# Autodesk Inventor assembly: BodyStructure
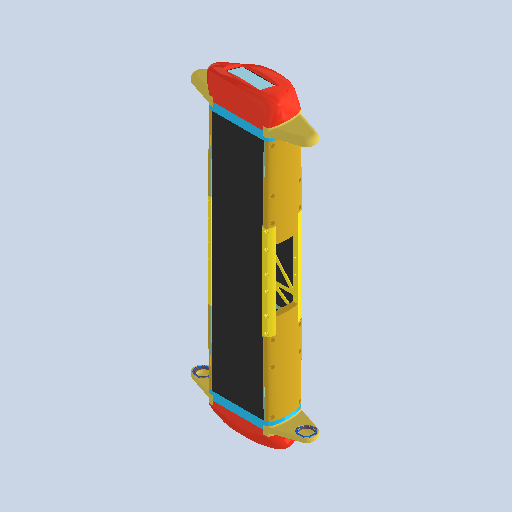
[picture p0: Inventor's stored thumbnail of the model, 512x512]
Saved by Autodesk Inventor 2023 (Build 270158000, 158)
## iProperties
Created: 2022-01-14
Part Number: BodyStructure
Document SubType Name: Assembly
Designer: Jochen
Author: Jochen
## Documents named in this file (11)
- D:\Projects\Lisbeth\CAD\BodyStructure.iam
- D:\Projects\Lisbeth\CAD\Body\BodyStructure Side.ipt
- D:\Projects\Lisbeth\CAD\Body\BodyStructure HipSupport.ipt
- D:\Projects\Lisbeth\CAD\Body\BodyStructure Centre Top.ipt
- D:\Projects\Lisbeth\CAD\Common\Bearing\bearing_27_20_4 s61704-2rsr.ipt
- D:\Projects\Lisbeth\CAD\Body\BodyCover.ipt
- D:\Projects\Lisbeth\CAD\Common\Accessories\Battery Pack.ipt
- D:\Projects\Lisbeth\CAD\Body\BodyStructure Head.ipt
- D:\Projects\Lisbeth\CAD\Body\BodyStructure Tail.ipt
- D:\Projects\Lisbeth\CAD\Common\Accessories\Adafruit 2.4 OLED display.ipt
- D:\Projects\Lisbeth\CAD\Body\BodyStructure Plate.ipt
## Components (24 placed, 9 different names)
1. BodyHipSupport:1 — Mate:38, Mate:39, Mate:230, Mate:231
2. BodyHipSupport:2 — Mate:44, Mate:45, Mate:226, Mate:227
3. BodyHipSupport:3 — Mate:42, Mate:43, Mate:188, Mate:189
4. BodyHipSupport:4 — Mate:40, Mate:41, Mate:147, Mate:148
5. bearing_27_20_4 s61704-2rsr:1 — Mate:38, Mate:39
6. bearing_27_20_4 s61704-2rsr:2 — Mate:44, Mate:45
7. bearing_27_20_4 s61704-2rsr:3 — Mate:40, Mate:41
8. bearing_27_20_4 s61704-2rsr:4 — Mate:42, Mate:43
9. BodyCover:1 — Mate:217, Mate:219
10. BodyCover:2 — Angle:1, Mate:202, Mate:204
11. Battery Pack 59x31x21:1 — Angle:1, Mate:159, Mate:222
12. BodyStructure Head:4 — Mate:147, Mate:148, Mate:159, Mate:185, Mate:186, Mate:187, Mate:188, Mate:189, Mate:220, Mate:221, Mate:222
13. Adafruit 2.4 OLED display:1 — Mate:220, Mate:221
14. BodyStructure Side:1 — Mate:177, Mate:180, Mate:190, Mate:191, Mate:232
15. BodyStructure Side:2 — Mate:184, Mate:185, Mate:186, Mate:213, Mate:233, Mate:235, Mate:236
16. BodyStructure Side:3 — Mate:181, Mate:187, Mate:234
17. BodyStructure Side:4 — Mate:192, Mate:193, Mate:194, Mate:208, Mate:212, Mate:228, Mate:229
18. Body Structure Centre Top:1 — Mate:180, Mate:207, Mate:208, Mate:211, Mate:218
19. Body Structure Centre Top:2 — Mate:177, Mate:181, Mate:184, Mate:212, Mate:213
20. Body Structure Centre:1 — Mate:190, Mate:191, Mate:192, Mate:202, Mate:204, Mate:232
21. Body Structure Centre:2 — Mate:193, Mate:194, Mate:217, Mate:218, Mate:219
22. Body Structure Centre:4 — Mate:234, Mate:235, Mate:236
23. Body Structure Centre:5 — Mate:207, Mate:211, Mate:233
24. BodyStructure Head:5 — Mate:226, Mate:227, Mate:228, Mate:229, Mate:230, Mate:231
## Relationships (50: Mate 49, Angle 1)
- Mate:38: BodyHipSupport:1 ↔ bearing_27_20_4 s61704-2rsr:1
- Mate:39: BodyHipSupport:1 ↔ bearing_27_20_4 s61704-2rsr:1
- Mate:40: BodyHipSupport:4 ↔ bearing_27_20_4 s61704-2rsr:3
- Mate:41: BodyHipSupport:4 ↔ bearing_27_20_4 s61704-2rsr:3
- Mate:42: BodyHipSupport:3 ↔ bearing_27_20_4 s61704-2rsr:4
- Mate:43: BodyHipSupport:3 ↔ bearing_27_20_4 s61704-2rsr:4
- Mate:44: BodyHipSupport:2 ↔ bearing_27_20_4 s61704-2rsr:2
- Mate:45: BodyHipSupport:2 ↔ bearing_27_20_4 s61704-2rsr:2
- Angle:1 (0 deg): BodyCover:2 ↔ Battery Pack 59x31x21:1
- Mate:147: BodyHipSupport:4 ↔ BodyStructure Head:4
- Mate:148: BodyHipSupport:4 ↔ BodyStructure Head:4
- Mate:159 (1 mm): Battery Pack 59x31x21:1 ↔ BodyStructure Head:4
- Mate:177: BodyStructure Side:1 ↔ Body Structure Centre Top:2
- Mate:180: BodyStructure Side:1 ↔ Body Structure Centre Top:1
- Mate:181: BodyStructure Side:3 ↔ Body Structure Centre Top:2
- Mate:184: BodyStructure Side:2 ↔ Body Structure Centre Top:2
- Mate:185: BodyStructure Head:4 ↔ BodyStructure Side:2
- Mate:186: BodyStructure Head:4 ↔ BodyStructure Side:2
- Mate:187: BodyStructure Head:4 ↔ BodyStructure Side:3
- Mate:188: BodyHipSupport:3 ↔ BodyStructure Head:4
- Mate:189: BodyHipSupport:3 ↔ BodyStructure Head:4
- Mate:190: BodyStructure Side:1 ↔ Body Structure Centre:1
- Mate:191: BodyStructure Side:1 ↔ Body Structure Centre:1
- Mate:192: BodyStructure Side:4 ↔ Body Structure Centre:1
- Mate:193: BodyStructure Side:4 ↔ Body Structure Centre:2
- Mate:194: BodyStructure Side:4 ↔ Body Structure Centre:2
- Mate:202: BodyCover:2 ↔ Body Structure Centre:1
- Mate:204 (0.25 mm): BodyCover:2 ↔ Body Structure Centre:1
- Mate:207: Body Structure Centre Top:1 ↔ Body Structure Centre:5
- Mate:208: BodyStructure Side:4 ↔ Body Structure Centre Top:1
- Mate:211: Body Structure Centre Top:1 ↔ Body Structure Centre:5
- Mate:212: BodyStructure Side:4 ↔ Body Structure Centre Top:2
- Mate:213: BodyStructure Side:2 ↔ Body Structure Centre Top:2
- Mate:217: BodyCover:1 ↔ Body Structure Centre:2
- Mate:218: Body Structure Centre Top:1 ↔ Body Structure Centre:2
- Mate:219: BodyCover:1 ↔ Body Structure Centre:2
- Mate:220: BodyStructure Head:4 ↔ Adafruit 2.4 OLED display:1
- Mate:221: BodyStructure Head:4 ↔ Adafruit 2.4 OLED display:1
- Mate:222 (0.5 mm): Battery Pack 59x31x21:1 ↔ BodyStructure Head:4
- Mate:226: BodyHipSupport:2 ↔ BodyStructure Head:5
- Mate:227: BodyHipSupport:2 ↔ BodyStructure Head:5
- Mate:228: BodyStructure Side:4 ↔ BodyStructure Head:5
- Mate:229: BodyStructure Side:4 ↔ BodyStructure Head:5
- Mate:230: BodyHipSupport:1 ↔ BodyStructure Head:5
- Mate:231: BodyHipSupport:1 ↔ BodyStructure Head:5
- Mate:232: BodyStructure Side:1 ↔ Body Structure Centre:1
- Mate:233: BodyStructure Side:2 ↔ Body Structure Centre:5
- Mate:234: BodyStructure Side:3 ↔ Body Structure Centre:4
- Mate:235: BodyStructure Side:2 ↔ Body Structure Centre:4
- Mate:236: BodyStructure Side:2 ↔ Body Structure Centre:4
